# Autodesk Inventor assembly: толстая+тонкая 2.0
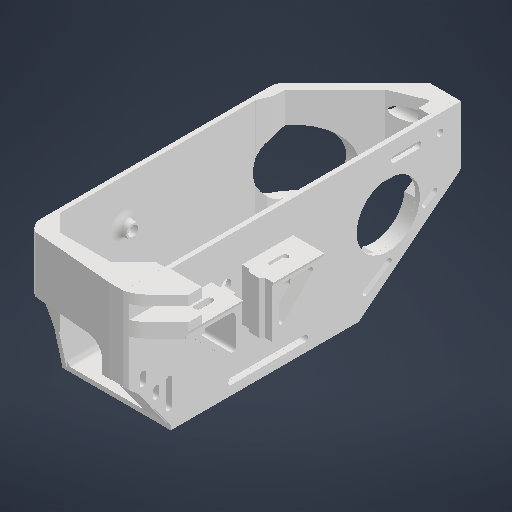
[picture p0: Inventor's stored thumbnail of the model, 512x512]
Saved by Autodesk Inventor 2025 (Build 290162000, 162)
## iProperties
Created: 2024-10-15
Part Number: толстая+тонкая 2.0
Document SubType Name: Assembly
Designer: Phantom
Author: Phantom
## Documents named in this file (3)
- C:\Users\GameHD\Desktop\Phantom 16950\толстая+тонкая 2.0.iam
- C:\Users\GameHD\Desktop\Phantom 16950\другая СОВЕРШЕННОЕ ТОНКАЯ.ipt
- C:\Users\GameHD\Desktop\Phantom 16950\другая СОВЕРШЕННОЕ ТОЛСТАЯ.ipt
## Components (2 placed, 2 different names)
1. другая СОВЕРШЕННОЕ ТОНКАЯ:1 — Совмещение:1, Заподлицо:1, Заподлицо:2
2. другая СОВЕРШЕННОЕ ТОЛСТАЯ:1 — Совмещение:1, Заподлицо:1, Заподлицо:2
## Relationships (3: Flush 2, Mate 1)
- Совмещение:1 [Mate]: другая СОВЕРШЕННОЕ ТОНКАЯ:1 ↔ другая СОВЕРШЕННОЕ ТОЛСТАЯ:1
- Заподлицо:1 [Flush]: другая СОВЕРШЕННОЕ ТОНКАЯ:1 ↔ другая СОВЕРШЕННОЕ ТОЛСТАЯ:1
- Заподлицо:2 [Flush]: другая СОВЕРШЕННОЕ ТОНКАЯ:1 ↔ другая СОВЕРШЕННОЕ ТОЛСТАЯ:1
